# Autodesk Inventor assembly: SQUICK_full
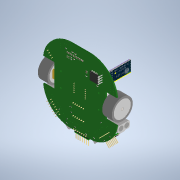
[picture p0: Inventor's stored thumbnail of the model, 180x180]
Saved by Autodesk Inventor 2020.3 (Build 243373000, 373)
## iProperties
Created: 2021-03-17
Part Number: SQUICK_full
Document SubType Name: Assembly
Designer: patry
Author: patry
## iProperties of the stored document 1x6 Male Pin Header.ipt
Created: 2018-11-15
Part Number: 1x6 Male Pin Header
Material: Ogólny
Description: STEP AP214
Document SubType Name: Modeling
Designer: patry
Density: 1 g/cm^3
Appearance: Domyślna
Preprocessor: SwSTEP 2.0
Title: 1x6 Male Pin Header.STEP
Author: M.B.I.
Revision Number: ANY
## Documents named in this file (18)
- C:\Users\patry\Desktop\MM Squick\squick_inventor\Workspace\SQUICK_full.iam
- C:\Users\patry\Desktop\MM Squick\squick_inventor\Workspace\Motor with brace\micro-metal-gearmotor-extended-with-1089-extended-bracket.ipt
- C:\Users\patry\Desktop\MM Squick\squick_inventor\Workspace\Encoders\magnetic-encoder-pair-kit-for-micro-metal-gearmotors-hpcb-compatible\magnetic-encoder-pair-kit-for-micro-metal-gearmotors-hpcb-compatible-enc0.ipt
- C:\Users\patry\Desktop\MM Squick\squick_inventor\Workspace\Encoders\magnetic-encoder-pair-kit-for-micro-metal-gearmotors-hpcb-compatible\magnetic-encoder-pair-kit-for-micro-metal-gearmotors-hpcb-compatible-w1r0.ipt
- C:\Users\patry\Desktop\MM Squick\squick_inventor\Workspace\PINS\GCT_BF02106AB04000280NG\AIS2020\BF021-06-A-B-0400-0280-N-G.iam
- C:\Users\patry\Desktop\MM Squick\squick_inventor\Workspace\BT_Module\BLUTOOTH.ipt
- C:\Users\patry\Desktop\MM Squick\squick_inventor\Workspace\Power\pololu-2843-step-down-regulator-5-volt-1.snapshot.2\Pololu 2843 5V Step Down Regulator.ipt
- C:\Users\patry\Desktop\MM Squick\squick_inventor\Workspace\PINS\single-row-male-pin-headers-1.snapshot.3\1x4 Male Pin Header Angle.ipt
- C:\Users\patry\Desktop\MM Squick\squick_inventor\Workspace\VL\vl53l0x-vl53l1x-vl53l3cx-carrier-model.ipt
- C:\Users\patry\Desktop\MM Squick\squick_inventor\Workspace\PINS\single-row-male-pin-headers-1.snapshot.3\1x7 Male Pin Header Angle.ipt
- C:\Users\patry\Desktop\MM Squick\squick_inventor\Workspace\Adafruit_IMU\Adafruit_IMU.ipt
- C:\Users\patry\Desktop\MM Squick\squick_inventor\Workspace\Kola\felga.ipt
- C:\Users\patry\Desktop\MM Squick\squick_inventor\Workspace\Kola\opona.ipt
- C:\Users\patry\Desktop\MM Squick\squick_inventor\Workspace\Board_base\KiCAD_board.iam
- **C:\Users\patry\Desktop\MM Squick\squick_inventor\Workspace\SQUICK_full.iam*LocalDocs*xAaaaaycaAaaaaaaaAaaaq2onTc*1x6 Male Pin Header.ipt
- C:\Users\patry\Desktop\MM Squick\squick_inventor\Workspace\Czujnik IR\obudowa.ipt
- C:\Users\patry\Desktop\MM Squick\squick_inventor\Workspace\Czujnik IR\obudowa_stand.ipt
- C:\Users\patry\Desktop\MM Squick\squick_inventor\Workspace\PINS\single-row-male-pin-headers-1.snapshot.3\1x6 Male Pin Header.STEP
## Components (30 placed, 16 different names)
1. micro-metal-gearmotor-extended-with-1089-extended-bracket:2 — Zestawiające:6, Zestawiające:10, Zestawiające:13, Zestawiające:41, Zestawiające:42, Zestawiające:43, Zestawiające:44, Równoległe:16, Kątowe:5
2. magnetic-encoder-pair-kit-for-micro-metal-gearmotors-hpcb-compatible-enc0:2 — Zestawiające:10, Zestawiające:11, Zestawiające:13, Zestawiające:22, Kątowe:4
3. magnetic-encoder-pair-kit-for-micro-metal-gearmotors-hpcb-compatible-w1r0:2 — Zestawiające:6, Zestawiające:11
4. BF021-06-A-B-0400-0280-N-G:1 [sub-assembly] — Zestawiające:59, Zestawiające:60
5. BLUTOOTH:1 — Zestawiające:47, Kątowe:1
6. Pololu 2843 5V Step Down Regulator:1 — Zestawiające:17, Równoległe:3, Równoległe:4, Zestawiające:67, Kątowe:11
7. 1x4 Male Pin Header Angle:1 — Zestawiające:17, Równoległe:3, Równoległe:4
8. BF021-06-A-B-0400-0280-N-G:2 [sub-assembly] — Zestawiające:22, Zestawiające:46
9. vl53l0x-vl53l1x-vl53l3cx-carrier-model:2 — Zestawiające:45, Kątowe:2
10. 1x7 Male Pin Header Angle:3
11. Adafruit_IMU:1 — Kątowe:8, Zestawiające:63, Zestawiające:64, Kątowe:9, Zestawiające:66, Kątowe:10
12. felga:1 — Zestawiające:33, Równoległe:13, Zestawiające:44, Równoległe:16, Kątowe:5
13. opona:1 — Zestawiające:33, Równoległe:13
14. KiCAD_board:1 [sub-assembly] — Zestawiające:41, Zestawiające:42, Zestawiające:43, Zestawiające:45, Zestawiające:46, Zestawiające:47, Kątowe:1, Kątowe:2, Zestawiające:49, Kątowe:3, Kątowe:4, Zestawiające:56, Zestawiające:57, Zestawiające:58, Zestawiające:59, Zestawiające:62, Kątowe:7, Kątowe:8, Zestawiające:63, Zestawiające:65, Zestawiające:67, Kątowe:11, Zestawiające:68, Kątowe:12, Zestawiające:69, Kątowe:13, Zestawiające:70, Kątowe:14, Zestawiające:71, Zestawiające:74
15. vl53l0x-vl53l1x-vl53l3cx-carrier-model:3 — Zestawiające:49, Kątowe:3
16. 1x7 Male Pin Header Angle:4
17. micro-metal-gearmotor-extended-with-1089-extended-bracket:3 — Zestawiające:56, Zestawiające:57, Zestawiające:58
18. magnetic-encoder-pair-kit-for-micro-metal-gearmotors-hpcb-compatible-enc0:3 — Zestawiające:60
19. magnetic-encoder-pair-kit-for-micro-metal-gearmotors-hpcb-compatible-w1r0:3
20. felga:2
21. opona:2
22. vl53l0x-vl53l1x-vl53l3cx-carrier-model:4 — Kątowe:7, Zestawiające:75
23. 1x7 Male Pin Header Angle:5 — Zestawiające:62
24. 1x6 Male Pin Header:1 — Zestawiające:64, Kątowe:9, Zestawiające:65
25. 1x6 Male Pin Header:2 — Zestawiające:66, Kątowe:10
26. obudowa:1 — Zestawiające:68, Kątowe:13
27. obudowa:2 — Kątowe:12, Zestawiające:69, Równoległe:21
28. obudowa:3 — Zestawiające:70, Kątowe:14
29. obudowa:4 — Zestawiające:71, Równoległe:21
30. obudowa_stand:2 — Zestawiające:74, Zestawiające:75
## Relationships (68: Mate 41, Angle 14, Flush 13)
- Zestawiające:6 [Mate]: micro-metal-gearmotor-extended-with-1089-extended-bracket:2 ↔ magnetic-encoder-pair-kit-for-micro-metal-gearmotors-hpcb-compatible-w1r0:2
- Zestawiające:10 [Mate]: micro-metal-gearmotor-extended-with-1089-extended-bracket:2 ↔ magnetic-encoder-pair-kit-for-micro-metal-gearmotors-hpcb-compatible-enc0:2
- Zestawiające:11 [Mate] (0.5 mm): magnetic-encoder-pair-kit-for-micro-metal-gearmotors-hpcb-compatible-enc0:2 ↔ magnetic-encoder-pair-kit-for-micro-metal-gearmotors-hpcb-compatible-w1r0:2
- Zestawiające:13 [Mate]: micro-metal-gearmotor-extended-with-1089-extended-bracket:2 ↔ magnetic-encoder-pair-kit-for-micro-metal-gearmotors-hpcb-compatible-enc0:2
- Zestawiające:17 [Mate]: Pololu 2843 5V Step Down Regulator:1 ↔ 1x4 Male Pin Header Angle:1
- Równoległe:3 [Flush]: Pololu 2843 5V Step Down Regulator:1 ↔ 1x4 Male Pin Header Angle:1
- Równoległe:4 [Flush] (0.15 mm): Pololu 2843 5V Step Down Regulator:1 ↔ 1x4 Male Pin Header Angle:1
- Zestawiające:22 [Mate]: magnetic-encoder-pair-kit-for-micro-metal-gearmotors-hpcb-compatible-enc0:2 ↔ BF021-06-A-B-0400-0280-N-G:2
- [Mate]: vl53l0x-vl53l1x-vl53l3cx-carrier-model:2 ↔ 1x7 Male Pin Header Angle:3
- [Flush]: vl53l0x-vl53l1x-vl53l3cx-carrier-model:2 ↔ 1x7 Male Pin Header Angle:3
- [Flush]: vl53l0x-vl53l1x-vl53l3cx-carrier-model:2 ↔ 1x7 Male Pin Header Angle:3
- Zestawiające:33 [Mate]: felga:1 ↔ opona:1
- Równoległe:13 [Flush]: felga:1 ↔ opona:1
- Zestawiające:41 [Mate]: micro-metal-gearmotor-extended-with-1089-extended-bracket:2 ↔ KiCAD_board:1
- Zestawiające:42 [Mate]: micro-metal-gearmotor-extended-with-1089-extended-bracket:2 ↔ KiCAD_board:1
- Zestawiające:43 [Mate]: micro-metal-gearmotor-extended-with-1089-extended-bracket:2 ↔ KiCAD_board:1
- Zestawiające:44 [Mate]: micro-metal-gearmotor-extended-with-1089-extended-bracket:2 ↔ felga:1
- Zestawiające:45 [Mate]: vl53l0x-vl53l1x-vl53l3cx-carrier-model:2 ↔ KiCAD_board:1
- Zestawiające:46 [Mate]: BF021-06-A-B-0400-0280-N-G:2 ↔ KiCAD_board:1
- Zestawiające:47 [Mate]: BLUTOOTH:1 ↔ KiCAD_board:1
- Kątowe:1 [Angle] (180 deg): BLUTOOTH:1 ↔ KiCAD_board:1
- Kątowe:2 [Angle] (225 deg): vl53l0x-vl53l1x-vl53l3cx-carrier-model:2 ↔ KiCAD_board:1
- [Mate]: vl53l0x-vl53l1x-vl53l3cx-carrier-model:3 ↔ 1x7 Male Pin Header Angle:4
- [Flush]: vl53l0x-vl53l1x-vl53l3cx-carrier-model:3 ↔ 1x7 Male Pin Header Angle:4
- [Flush]: vl53l0x-vl53l1x-vl53l3cx-carrier-model:3 ↔ 1x7 Male Pin Header Angle:4
- Zestawiające:49 [Mate]: KiCAD_board:1 ↔ vl53l0x-vl53l1x-vl53l3cx-carrier-model:3
- Kątowe:3 [Angle] (0 deg): KiCAD_board:1 ↔ vl53l0x-vl53l1x-vl53l3cx-carrier-model:3
- Kątowe:4 [Angle] (180 deg): magnetic-encoder-pair-kit-for-micro-metal-gearmotors-hpcb-compatible-enc0:2 ↔ KiCAD_board:1
- Równoległe:16 [Flush]: micro-metal-gearmotor-extended-with-1089-extended-bracket:2 ↔ felga:1
- Kątowe:5 [Angle] (180 deg): micro-metal-gearmotor-extended-with-1089-extended-bracket:2 ↔ felga:1
- [Mate]: micro-metal-gearmotor-extended-with-1089-extended-bracket:3 ↔ magnetic-encoder-pair-kit-for-micro-metal-gearmotors-hpcb-compatible-w1r0:3
- [Mate]: micro-metal-gearmotor-extended-with-1089-extended-bracket:3 ↔ magnetic-encoder-pair-kit-for-micro-metal-gearmotors-hpcb-compatible-enc0:3
- [Mate] (0.5 mm): magnetic-encoder-pair-kit-for-micro-metal-gearmotors-hpcb-compatible-enc0:3 ↔ magnetic-encoder-pair-kit-for-micro-metal-gearmotors-hpcb-compatible-w1r0:3
- [Mate]: micro-metal-gearmotor-extended-with-1089-extended-bracket:3 ↔ magnetic-encoder-pair-kit-for-micro-metal-gearmotors-hpcb-compatible-enc0:3
- [Mate]: felga:2 ↔ opona:2
- [Flush]: felga:2 ↔ opona:2
- [Mate]: micro-metal-gearmotor-extended-with-1089-extended-bracket:3 ↔ felga:2
- [Flush]: micro-metal-gearmotor-extended-with-1089-extended-bracket:3 ↔ felga:2
- [Angle] (180 deg): micro-metal-gearmotor-extended-with-1089-extended-bracket:3 ↔ felga:2
- Zestawiające:56 [Mate]: KiCAD_board:1 ↔ micro-metal-gearmotor-extended-with-1089-extended-bracket:3
- Zestawiające:57 [Mate]: KiCAD_board:1 ↔ micro-metal-gearmotor-extended-with-1089-extended-bracket:3
- Zestawiające:58 [Mate]: KiCAD_board:1 ↔ micro-metal-gearmotor-extended-with-1089-extended-bracket:3
- Zestawiające:59 [Mate]: BF021-06-A-B-0400-0280-N-G:1 ↔ KiCAD_board:1
- Zestawiające:60 [Mate]: BF021-06-A-B-0400-0280-N-G:1 ↔ magnetic-encoder-pair-kit-for-micro-metal-gearmotors-hpcb-compatible-enc0:3
- [Mate]: vl53l0x-vl53l1x-vl53l3cx-carrier-model:4 ↔ 1x7 Male Pin Header Angle:5
- [Flush]: vl53l0x-vl53l1x-vl53l3cx-carrier-model:4 ↔ 1x7 Male Pin Header Angle:5
- [Flush]: vl53l0x-vl53l1x-vl53l3cx-carrier-model:4 ↔ 1x7 Male Pin Header Angle:5
- Zestawiające:62 [Mate]: KiCAD_board:1 ↔ 1x7 Male Pin Header Angle:5
- Kątowe:7 [Angle] (-45 deg): KiCAD_board:1 ↔ vl53l0x-vl53l1x-vl53l3cx-carrier-model:4
- Kątowe:8 [Angle] (0 deg): Adafruit_IMU:1 ↔ KiCAD_board:1
- Zestawiające:63 [Mate]: Adafruit_IMU:1 ↔ KiCAD_board:1
- Zestawiające:64 [Mate]: Adafruit_IMU:1 ↔ 1x6 Male Pin Header:1
- Kątowe:9 [Angle] (0 deg): Adafruit_IMU:1 ↔ 1x6 Male Pin Header:1
- Zestawiające:65 [Mate] (0.6 mm): KiCAD_board:1 ↔ 1x6 Male Pin Header:1
- Zestawiające:66 [Mate]: Adafruit_IMU:1 ↔ 1x6 Male Pin Header:2
- Kątowe:10 [Angle] (0 deg): Adafruit_IMU:1 ↔ 1x6 Male Pin Header:2
- Zestawiające:67 [Mate]: Pololu 2843 5V Step Down Regulator:1 ↔ KiCAD_board:1
- Kątowe:11 [Angle] (-45 deg): Pololu 2843 5V Step Down Regulator:1 ↔ KiCAD_board:1
- Zestawiające:68 [Mate]: KiCAD_board:1 ↔ obudowa:1
- Kątowe:12 [Angle] (0 deg): KiCAD_board:1 ↔ obudowa:2
- Zestawiające:69 [Mate]: KiCAD_board:1 ↔ obudowa:2
- Kątowe:13 [Angle] (-45 deg): KiCAD_board:1 ↔ obudowa:1
- Zestawiające:70 [Mate]: KiCAD_board:1 ↔ obudowa:3
- Kątowe:14 [Angle] (-45 deg): KiCAD_board:1 ↔ obudowa:3
- Zestawiające:71 [Mate]: KiCAD_board:1 ↔ obudowa:4
- Równoległe:21 [Flush]: obudowa:2 ↔ obudowa:4
- Zestawiające:74 [Mate]: KiCAD_board:1 ↔ obudowa_stand:2
- Zestawiające:75 [Mate] (5 mm): vl53l0x-vl53l1x-vl53l3cx-carrier-model:4 ↔ obudowa_stand:2
## Named parameters: d44_d39 = 0 mm, d45_d40 = 0 mm, d46_d41 = 0 mm, d90_d44_d39 = 0 mm, d91_d45_d40 = 0 mm, d92_d46_d41 = 0 mm, d98_d96 = 0 mm, d99_d97 = 180 deg, d100_d84 = 0 mm, d101_d78 = 0 mm, d102_d62 = 0 mm, d103_d7 = 0 mm, d104_d12 = 0 mm, d105_d14 = 0.5 mm, d106_d16 = 0 mm, d112_d90_d44_d39 = 0 mm, d113_d91_d45_d40 = 0 mm, d114_d92_d46_d41 = 0 mm
